# Autodesk Inventor assembly: combination
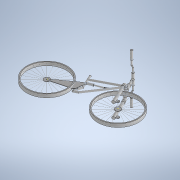
[picture p0: Inventor's stored thumbnail of the model, 180x180]
Saved by Autodesk Inventor 2020 (Build 240168000, 168)
## iProperties
Created: 2021-05-21
Part Number: combination
Document SubType Name: Assembly
Designer: 林昱秀
Author: 林昱秀
## Documents named in this file (11)
- E:\4072pj3\project3\40723102\Firebird 29 bike\combination.iam
- E:\4072pj3\project3\40723102\Firebird 29 bike\Frame.ipt
- E:\4072pj3\project3\40723102\Firebird 29 bike\Binary link.ipt
- E:\4072pj3\project3\40723102\Firebird 29 bike\Triangle link.ipt
- E:\4072pj3\project3\40723102\Firebird 29 bike\Binary link47.ipt
- E:\4072pj3\project3\40723102\Firebird 29 bike\Wheel.ipt
- E:\4072pj3\project3\40723102\Firebird 29 bike\Slider.ipt
- E:\4072pj3\project3\40723102\Firebird 29 bike\Slider1.ipt
- E:\4072pj3\project3\40723102\Firebird 29 bike\Fork.ipt
- E:\4072pj3\project3\40723102\Firebird 29 bike\pin.ipt
- E:\4072pj3\project3\40723102\Firebird 29 bike\Handlebar.ipt
## Components (11 placed, 10 different names)
1. Frame:1 — 角度:1, 貼合:1, 貼合:4, 貼合:7, 圓柱:2
2. Binary link:1 — 角度:2, 貼合:1, 貼合:2
3. Triangle link:1 — 角度:3, 貼合:2, 角度:4, 貼合:3, 貼合:5, 貼合:6, 角度:9
4. Binary link47:1 — 角度:4, 貼合:3, 貼合:4
5. Wheel:1 — 角度:5, 貼合:5
6. Slider:1 — 角度:6, 貼合:6, 圓柱:1
7. Slider1:1 — 角度:7, 貼合:7, 圓柱:1
8. Fork:1 — 角度:8, 圓柱:2, 貼合:8, 圓柱:3
9. Wheel:2 — 角度:10, 貼合:9
10. pin:1 — 角度:9, 貼合:8, 貼合:9
11. Handlebar:1 — 角度:11, 圓柱:3
## Relationships (23: Angle 11, Mate 9, CylindricalJoint 3)
- 角度:1 [Angle] (0 deg): Frame:1
- 角度:2 [Angle] (0 deg): Binary link:1
- 貼合:1 [Mate]: Frame:1 ↔ Binary link:1
- 角度:3 [Angle] (0 deg): Triangle link:1
- 貼合:2 [Mate]: Binary link:1 ↔ Triangle link:1
- 角度:4 [Angle] (0 deg): Triangle link:1 ↔ Binary link47:1
- 貼合:3 [Mate]: Triangle link:1 ↔ Binary link47:1
- 貼合:4 [Mate]: Frame:1 ↔ Binary link47:1
- 角度:5 [Angle] (0 deg): Wheel:1
- 貼合:5 [Mate]: Triangle link:1 ↔ Wheel:1
- 角度:6 [Angle] (0 deg): Slider:1
- 貼合:6 [Mate]: Triangle link:1 ↔ Slider:1
- 角度:7 [Angle] (0 deg): Slider1:1
- 貼合:7 [Mate]: Frame:1 ↔ Slider1:1
- 圓柱:1 [CylindricalJoint]: Slider:1 ↔ Slider1:1
- 角度:8 [Angle] (0 deg): Fork:1
- 圓柱:2 [CylindricalJoint]: Frame:1 ↔ Fork:1
- 角度:9 [Angle] (0 deg): Triangle link:1 ↔ pin:1
- 貼合:8 [Mate]: Fork:1 ↔ pin:1
- 角度:10 [Angle] (0 deg): Wheel:2
- 貼合:9 [Mate]: Wheel:2 ↔ pin:1
- 角度:11 [Angle] (0 deg): Handlebar:1
- 圓柱:3 [CylindricalJoint]: Fork:1 ↔ Handlebar:1
